# Autodesk Inventor assembly: HipLeftNCS
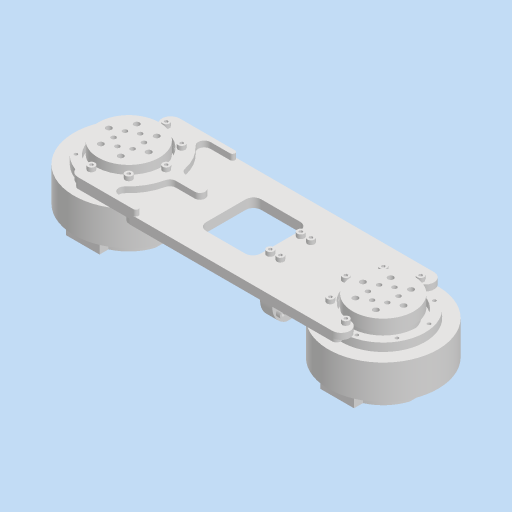
[picture p0: Inventor's stored thumbnail of the model, 512x512]
Saved by Autodesk Inventor 2023 (Build 270158000, 158)
## iProperties
Created: 2026-06-18
Part Number: HipLeftNCS
Document SubType Name: Assembly
Designer: Nathann
Author: Nathann
## Documents named in this file (2)
- C:\Users\Nathann\ClawdDrive\Objet3D\RunningRobot\PartURDF\HipLeftNCS.iam
- C:\Users\Nathann\ClawdDrive\Objet3D\RunningRobot\PartURDF\HipLeft_Simplify_1.ipt
## Components (1 placed, 1 different names)
1. HipLeft_Simplify_1:1 — Mate:1, Mate:2, Angle:1
## Relationships (5: Mate 4, Angle 1)
- Mate:1: HipLeft_Simplify_1:1
- Mate:2: HipLeft_Simplify_1:1
- Mate:3
- Mate:4
- Angle:1 (0 deg): HipLeft_Simplify_1:1
